# Autodesk Inventor assembly: Sessao5
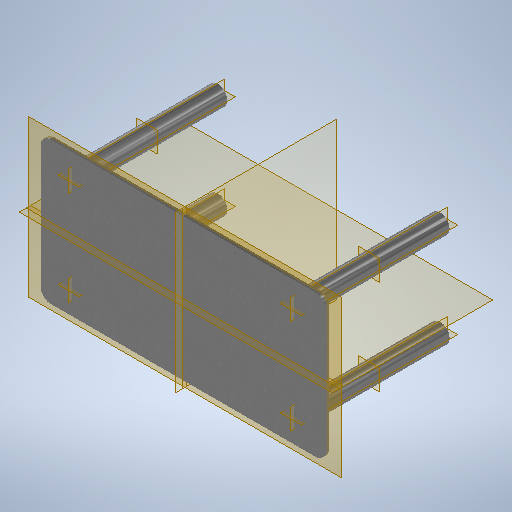
[picture p0: Inventor's stored thumbnail of the model, 512x512]
Saved by Autodesk Inventor 2025.2 (Build 292293000, 293)
## iProperties
Created: 2025-03-28
Part Number: Sessao5
Document SubType Name: Assembly
Designer: lucas
Author: lucas
## Documents named in this file (3)
- C:\Users\lucas\OneDrive\Documentos\Documentos\Gustavo\Mozangao\Robotica_Fundamentos\Inventor\Sessao5\Sessao5.iam
- C:\Users\lucas\OneDrive\Documentos\Documentos\Gustavo\Mozangao\Robotica_Fundamentos\Inventor\Sessao5\Sessao5_0001_001.ipt
- C:\Users\lucas\OneDrive\Documentos\Documentos\Gustavo\Mozangao\Robotica_Fundamentos\Inventor\Sessao5\Sessao5_0002_001.ipt
## Components (5 placed, 2 different names)
1. Sessao5_0001_001:1 — Alinhado:1, Alinhado:2, Alinhado:3, Coincidente:1
2. Sessao5_0002_001:1 — Alinhado:7, Alinhado:10, Alinhado:11, Simetria:1
3. Sessao5_0002_001:2 — Alinhado:6, Alinhado:9, Simetria:1
4. Sessao5_0002_001:3 — Alinhado:8, Alinhado:10, Simetria:2, Simetria:3
5. Sessao5_0002_001:4 — Coincidente:1, Alinhado:4, Alinhado:5, Alinhado:6, Alinhado:7, Alinhado:8, Alinhado:9, Alinhado:11, Simetria:2, Simetria:3
## Relationships (15: Flush 11, Symmetry 3, Mate 1)
- Alinhado:1 [Flush]: Sessao5_0001_001:1
- Alinhado:2 [Flush]: Sessao5_0001_001:1
- Alinhado:3 [Flush]: Sessao5_0001_001:1
- Coincidente:1 [Mate]: Sessao5_0001_001:1 ↔ Sessao5_0002_001:4
- Alinhado:4 [Flush] (586 mm): Sessao5_0002_001:4
- Alinhado:5 [Flush] (250 mm): Sessao5_0002_001:4
- Alinhado:6 [Flush]: Sessao5_0002_001:2 ↔ Sessao5_0002_001:4
- Alinhado:7 [Flush]: Sessao5_0002_001:1 ↔ Sessao5_0002_001:4
- Alinhado:8 [Flush]: Sessao5_0002_001:3 ↔ Sessao5_0002_001:4
- Alinhado:9 [Flush]: Sessao5_0002_001:2 ↔ Sessao5_0002_001:4
- Alinhado:10 [Flush]: Sessao5_0002_001:1 ↔ Sessao5_0002_001:3
- Alinhado:11 [Flush]: Sessao5_0002_001:1 ↔ Sessao5_0002_001:4
- Simetria:1 [Symmetry]: Sessao5_0002_001:1 ↔ Sessao5_0002_001:2
- Simetria:2 [Symmetry]: Sessao5_0002_001:3 ↔ Sessao5_0002_001:4
- Simetria:3 [Symmetry]: Sessao5_0002_001:3 ↔ Sessao5_0002_001:4
